# Autodesk Inventor assembly: funnel
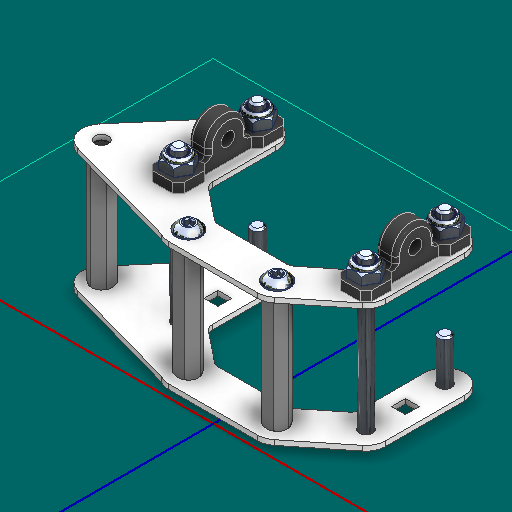
[picture p0: Inventor's stored thumbnail of the model, 512x512]
Saved by Autodesk Inventor 2025 (Build 290162000, 162)
## iProperties
Created: 2024-08-16
Part Number: funnel
Document SubType Name: Assembly
Designer: averey
Author: averey
## Documents named in this file (12)
- C:\Users\avere\vex_robotics_high_stakes\hardware\cad\ATLAS\chassis\drive_pod\funnel.iam
- C:\Users\avere\vex_robotics_high_stakes\hardware\cad\ATLAS\chassis\drive_pod\custom_parts\funnel_gusset.ipt
- C:\Users\avere\vex_robotics_high_stakes\hardware\cad\VEX-CAD-Inventor\Structure\Standoff\Standoff 1.50.ipt
- C:\Users\avere\vex_robotics_high_stakes\hardware\cad\VEX-CAD-Inventor\Structure\Standoff.ipt
- C:\Users\avere\vex_robotics_high_stakes\hardware\cad\VEX-CAD-Inventor\Structure\Hardware\Screw Steel - Star\SScrew Star Smooth .290.ipt
- C:\Users\avere\vex_robotics_high_stakes\hardware\cad\VEX-CAD-Inventor\Structure\Hardware\Screw Steel - Star.ipt
- C:\Users\avere\vex_robotics_high_stakes\hardware\cad\VEX-CAD-Inventor\Structure\Hardware\Screw Shoulder Robosource\SScrew Shoulder Smooth 2.000 x .04.ipt
- C:\Users\avere\vex_robotics_high_stakes\hardware\cad\VEX-CAD-Inventor\Structure\Hardware\Screw Shoulder Robosource.ipt
- C:\Users\avere\vex_robotics_high_stakes\hardware\cad\VEX-CAD-Inventor\Motion\Shaft LS\LS Pillow Bearing Block.ipt
- C:\Users\avere\vex_robotics_high_stakes\hardware\cad\VEX-CAD-Inventor\Structure\Hardware\Nut Thin Nylock.ipt
- C:\Users\avere\vex_robotics_high_stakes\hardware\cad\VEX-CAD-Inventor\Structure\Hardware\Screw Shoulder Robosource\SScrew Shoulder Smooth .500 x .18.ipt
- C:\Users\avere\vex_robotics_high_stakes\hardware\cad\VEX-CAD-Inventor\Structure\Hardware\Screw Steel - Star\SScrew Star Smooth .625.ipt
## Components (21 placed, 8 different names)
1. funnel_gusset:1 — Flush:1, Mate:3, Insert:11, Insert:13, Insert:14, Insert:16, Insert:20
2. funnel_gusset:2 — Insert:9, Insert:18, Insert:19
3. Standoff 1.50:1
4. Standoff 1.50:2 — Insert:9
5. SScrew Star Smooth .290:1
6. SScrew Star Smooth .290:2
7. SScrew Star Smooth .290:3
8. SScrew Star Smooth .290:4
9. SScrew Shoulder Smooth 2.000 x .04:1 — Mate:5
10. SScrew Shoulder Smooth 2.000 x .04:2 — Mate:4
11. LS Pillow Bearing Block:1 — Insert:11, Insert:15
12. Nut Thin Nylock:1 — Mate:4
13. LS Pillow Bearing Block:2 — Insert:13, Insert:17
14. Nut Thin Nylock:2 — Mate:5
15. Nut Thin Nylock:3 — Insert:15
16. SScrew Shoulder Smooth .500 x .18:3 — Insert:14
17. Nut Thin Nylock:4 — Insert:17
18. SScrew Shoulder Smooth .500 x .18:4 — Insert:16
19. SScrew Star Smooth .625:5 — Insert:19
20. SScrew Star Smooth .625:6 — Insert:18
21. Standoff 1.50:3 — Insert:20
## Relationships (26: Insert 20, Mate 5, Flush 1)
- [Mate]: funnel_gusset:1 ↔ funnel_gusset:2
- [Mate]: funnel_gusset:1 ↔ funnel_gusset:2
- [Insert]: funnel_gusset:1 ↔ Standoff 1.50:2
- [Insert]: funnel_gusset:1 ↔ Standoff 1.50:1
- [Insert]: funnel_gusset:1 ↔ SScrew Star Smooth .290:1
- [Insert]: funnel_gusset:1 ↔ SScrew Star Smooth .290:2
- [Insert]: funnel_gusset:2 ↔ SScrew Star Smooth .290:4
- [Insert]: funnel_gusset:2 ↔ SScrew Star Smooth .290:3
- [Insert]: funnel_gusset:2 ↔ SScrew Shoulder Smooth 2.000 x .04:1
- [Insert]: funnel_gusset:2 ↔ SScrew Shoulder Smooth 2.000 x .04:2
- Flush:1: funnel_gusset:1
- Insert:9: funnel_gusset:2 ↔ Standoff 1.50:2
- Mate:3 (23.8125 mm): funnel_gusset:1
- [Insert]: LS Pillow Bearing Block:1 ↔ Nut Thin Nylock:1
- Insert:11: funnel_gusset:1 ↔ LS Pillow Bearing Block:1
- Mate:4: SScrew Shoulder Smooth 2.000 x .04:2 ↔ Nut Thin Nylock:1
- [Insert]: LS Pillow Bearing Block:2 ↔ Nut Thin Nylock:2
- Insert:13: funnel_gusset:1 ↔ LS Pillow Bearing Block:2
- Mate:5: SScrew Shoulder Smooth 2.000 x .04:1 ↔ Nut Thin Nylock:2
- Insert:14 (1.5875 mm): funnel_gusset:1 ↔ SScrew Shoulder Smooth .500 x .18:3
- Insert:15: LS Pillow Bearing Block:1 ↔ Nut Thin Nylock:3
- Insert:16 (1.5875 mm): funnel_gusset:1 ↔ SScrew Shoulder Smooth .500 x .18:4
- Insert:17: LS Pillow Bearing Block:2 ↔ Nut Thin Nylock:4
- Insert:18: funnel_gusset:2 ↔ SScrew Star Smooth .625:6
- Insert:19: funnel_gusset:2 ↔ SScrew Star Smooth .625:5
- Insert:20: funnel_gusset:1 ↔ Standoff 1.50:3
## Named parameters: d16_d62 = 0 mm
